# Autodesk Inventor assembly: [总]惯性筛总装配
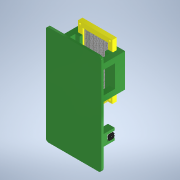
[picture p0: Inventor's stored thumbnail of the model, 180x180]
Saved by Autodesk Inventor 2022 (Build 260153000, 153)
## iProperties
Created: 2022-05-21
Part Number: [总]惯性筛总装配
Document SubType Name: Assembly
Designer: zhcne
Author: zhcne
## Documents named in this file (5)
- E:\Engineering_Development\SchoolProjects\2022_5_18_惯性筛_机电一体化课程设计\inertiascreen_curriculumdesign\3.Model\2.3D_Simulation\[总]惯性筛总装配.iam
- E:\Engineering_Development\SchoolProjects\2022_5_18_惯性筛_机电一体化课程设计\inertiascreen_curriculumdesign\3.Model\2.3D_Simulation\惯性筛筛网装配.iam
- E:\Engineering_Development\SchoolProjects\2022_5_18_惯性筛_机电一体化课程设计\inertiascreen_curriculumdesign\3.Model\2.3D_Simulation\惯性筛偏心轮装配.iam
- E:\Engineering_Development\SchoolProjects\2022_5_18_惯性筛_机电一体化课程设计\inertiascreen_curriculumdesign\3.Model\2.3D_Simulation\Ipt\4.机架\机架.ipt
- E:\Engineering_Development\SchoolProjects\2022_5_18_惯性筛_机电一体化课程设计\inertiascreen_curriculumdesign\3.Model\2.3D_Simulation\Ipt\2.轴承\ISO 1224 - 38 3 x  7 x  3.ipt
## Components (4 placed, 4 different names)
1. 惯性筛筛网装配:1 [sub-assembly] — 配合:1, 配合:2, 配合:4, 配合:5, 配合:6
2. 惯性筛偏心轮装配:1 [sub-assembly] — 配合:1, 配合:2, 配合:3, 表面齐平:1, 配合:9
3. 机架:1 — 配合:5, 配合:6, 表面齐平:1, 配合:7, 配合:8, 配合:9
4. UNI ISO 1224 (mm) 38 3 x  7 x  3:1 — 配合:7, 配合:8
## Relationships (10: Mate 9, Flush 1)
- 配合:1 [Mate] (4 mm): 惯性筛筛网装配:1 ↔ 惯性筛偏心轮装配:1
- 配合:2 [Mate]: 惯性筛筛网装配:1 ↔ 惯性筛偏心轮装配:1
- 配合:3 [Mate]: 惯性筛偏心轮装配:1
- 配合:4 [Mate]: 惯性筛筛网装配:1
- 配合:5 [Mate] (0.5 mm): 惯性筛筛网装配:1 ↔ 机架:1
- 配合:6 [Mate] (0.5 mm): 惯性筛筛网装配:1 ↔ 机架:1
- 表面齐平:1 [Flush] (22 mm): 惯性筛偏心轮装配:1 ↔ 机架:1
- 配合:7 [Mate]: 机架:1 ↔ UNI ISO 1224 (mm) 38 3 x  7 x  3:1
- 配合:8 [Mate]: 机架:1 ↔ UNI ISO 1224 (mm) 38 3 x  7 x  3:1
- 配合:9 [Mate] (0.5 mm): 惯性筛偏心轮装配:1 ↔ 机架:1
